# Autodesk Inventor assembly: idler
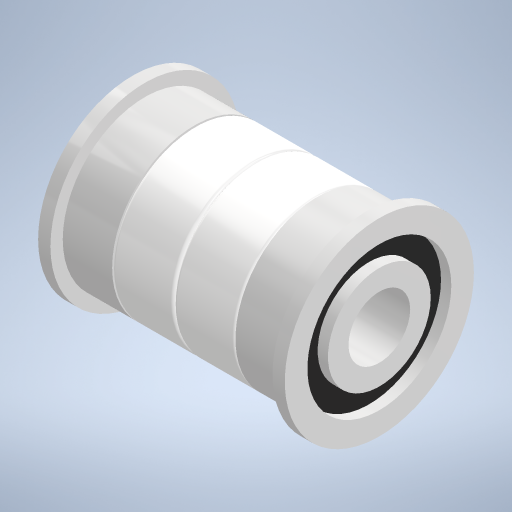
[picture p0: Inventor's stored thumbnail of the model, 512x512]
Saved by Autodesk Inventor 2023 (Build 270158000, 158)
## iProperties
Created: 2022-06-28
Part Number: idler
Document SubType Name: Assembly
Designer: user
Author: user
## Documents named in this file (3)
- C:\Users\user\Desktop\V-core-3-main\model\V-core 3 idex\v3\machine file\idler.iam
- C:\Users\user\Desktop\V-core-3-main\model\V-core 3 idex\v3\machine file\MF83ZZ-Bearing.ipt
- C:\Users\user\Desktop\V-core-3-main\model\V-core 3 idex\v3\machine file\MR83-2Z - Deep groove ball bearing.ipt
## Components (4 placed, 2 different names)
1. MF83ZZ-Bearing:1 — 貼合:1, 貼合:2
2. MR83-2Z - Deep groove ball bearing:1 — 貼合:1, 貼合:2, 貼合:3, 貼合:4
3. MF83ZZ-Bearing:2 — 貼合:5, 貼合:6
4. MR83-2Z - Deep groove ball bearing:2 — 貼合:3, 貼合:4, 貼合:5, 貼合:6
## Relationships (6: Mate 6)
- 貼合:1 [Mate]: MF83ZZ-Bearing:1 ↔ MR83-2Z - Deep groove ball bearing:1
- 貼合:2 [Mate]: MF83ZZ-Bearing:1 ↔ MR83-2Z - Deep groove ball bearing:1
- 貼合:3 [Mate]: MR83-2Z - Deep groove ball bearing:1 ↔ MR83-2Z - Deep groove ball bearing:2
- 貼合:4 [Mate]: MR83-2Z - Deep groove ball bearing:1 ↔ MR83-2Z - Deep groove ball bearing:2
- 貼合:5 [Mate]: MF83ZZ-Bearing:2 ↔ MR83-2Z - Deep groove ball bearing:2
- 貼合:6 [Mate]: MF83ZZ-Bearing:2 ↔ MR83-2Z - Deep groove ball bearing:2
